# Autodesk Inventor assembly: Telaietto trasmissione - Taglio
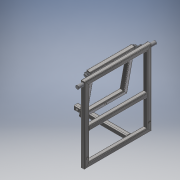
[picture p0: Inventor's stored thumbnail of the model, 180x180]
Saved by Autodesk Inventor 2018 (Build 220112000, 112)
## iProperties
Created: 2020-06-04
Part Number: Telaietto trasmissione - Taglio
Material: Generico
Document SubType Name: Weldment
Designer: Francesco
Weld Material: Welded Aluminum-6061
Mass: 1931.15 g
Surface Area: 2480.54 cm^2
Volume: 246.006 cm^3
Density: 7.85 g/cm^3
Author: Francesco
## Documents named in this file (10)
- C:\Users\Francesco\no-brim\Meccanica\Progetto Inventor no-brim\Assiemi\Telaietto trasmissione - Taglio.iam
- C:\Users\Francesco\no-brim\Meccanica\Progetto Inventor no-brim\Parti\Tubolare telaietto corto.ipt
- C:\Users\Francesco\no-brim\Meccanica\Progetto Inventor no-brim\Parti\Tubolare telaietto lungo 45.ipt
- C:\Users\Francesco\no-brim\Meccanica\Progetto Inventor no-brim\Parti\Tubolare telaietto corto 45.ipt
- C:\Users\Francesco\no-brim\Meccanica\Progetto Inventor no-brim\Parti\Tubolare telaietto corto 45 motore.ipt
- C:\Users\Francesco\no-brim\Meccanica\Progetto Inventor no-brim\Parti\Tubolare telaietto corto 45 motore per perni.ipt
- C:\Users\Francesco\no-brim\Meccanica\Progetto Inventor no-brim\Parti\Perno tendi motore.ipt
- C:\Users\Francesco\no-brim\Meccanica\Progetto Inventor no-brim\Parti\Supporto perno tendi motore.ipt
- C:\Users\Francesco\no-brim\Meccanica\Progetto Inventor no-brim\Parti\Perno movimento lama.ipt
- C:\Users\Francesco\no-brim\Meccanica\Progetto Inventor no-brim\Parti\Tubolare telaietto verticale.ipt
## Components (17 placed, 6 different names)
1. Tubolare telaietto corto:2 — Coincidente:8, Allineato:5, Coincidente:9
2. Tubolare telaietto lungo 45:1 — Coincidente:1, Allineato:1, Coincidente:2, Coincidente:5, Allineato:3, Coincidente:6, Coincidente:8, Allineato:5, Angolo:1, Coincidente:50, Coincidente:51, Allineato:20
3. Tubolare telaietto lungo 45:2 — Coincidente:3, Allineato:2, Coincidente:4, Allineato:18, Coincidente:48, Coincidente:49
4. Tubolare telaietto corto:3 — Coincidente:1, Allineato:1, Coincidente:2, Coincidente:3, Allineato:2, Coincidente:4, Coincidente:9, Coincidente:27, Coincidente:31, Allineato:14
5. Tubolare telaietto corto:4 — Coincidente:5, Allineato:3, Coincidente:6, Coincidente:52, Allineato:19
6. Perno tendi motore:1 — Coincidente:34, Coincidente:41
7. Perno tendi motore:2 — Coincidente:33, Coincidente:42, Coincidente:43
8. Supporto perno tendi motore:1 — Coincidente:31, Coincidente:33, Allineato:14, Coincidente:44
9. Supporto perno tendi motore:2 — Coincidente:27, Coincidente:34, Coincidente:47, Allineato:18
10. Tubolare telaietto corto:11 — Coincidente:35, Coincidente:36, Allineato:15, Coincidente:39, Allineato:17, Coincidente:40
11. Tubolare telaietto corto:12 — Coincidente:37, Allineato:16, Coincidente:38
12. Tubolare telaietto corto:13 — Coincidente:39, Allineato:17, Coincidente:40, Coincidente:45, Coincidente:46, Coincidente:47
13. Tubolare telaietto corto:14 — Coincidente:35, Coincidente:36, Allineato:15, Coincidente:37, Allineato:16, Coincidente:38, Coincidente:41, Coincidente:42, Coincidente:43, Coincidente:44, Angolo:1
14. Perno tendi motore:3 — Coincidente:45, Coincidente:46
15. Perno movimento lama:1 — Coincidente:48, Coincidente:49
16. Perno movimento lama:2 — Coincidente:50, Coincidente:51
17. Tubolare telaietto verticale:1 — Coincidente:52, Allineato:19, Allineato:20
## Relationships (42: Mate 30, Flush 11, Angle 1)
- Coincidente:1 [Mate]: Tubolare telaietto lungo 45:1 ↔ Tubolare telaietto corto:3
- Allineato:1 [Flush]: Tubolare telaietto lungo 45:1 ↔ Tubolare telaietto corto:3
- Coincidente:2 [Mate]: Tubolare telaietto lungo 45:1 ↔ Tubolare telaietto corto:3
- Coincidente:3 [Mate]: Tubolare telaietto lungo 45:2 ↔ Tubolare telaietto corto:3
- Allineato:2 [Flush]: Tubolare telaietto lungo 45:2 ↔ Tubolare telaietto corto:3
- Coincidente:4 [Mate]: Tubolare telaietto lungo 45:2 ↔ Tubolare telaietto corto:3
- Coincidente:5 [Mate]: Tubolare telaietto lungo 45:1 ↔ Tubolare telaietto corto:4
- Allineato:3 [Flush]: Tubolare telaietto lungo 45:1 ↔ Tubolare telaietto corto:4
- Coincidente:6 [Mate]: Tubolare telaietto lungo 45:1 ↔ Tubolare telaietto corto:4
- Coincidente:8 [Mate]: Tubolare telaietto corto:2 ↔ Tubolare telaietto lungo 45:1
- Allineato:5 [Flush]: Tubolare telaietto corto:2 ↔ Tubolare telaietto lungo 45:1
- Coincidente:9 [Mate] (-200 mm): Tubolare telaietto corto:2 ↔ Tubolare telaietto corto:3
- Coincidente:27 [Mate]: Tubolare telaietto corto:3 ↔ Supporto perno tendi motore:2
- Coincidente:31 [Mate]: Tubolare telaietto corto:3 ↔ Supporto perno tendi motore:1
- Coincidente:33 [Mate]: Perno tendi motore:2 ↔ Supporto perno tendi motore:1
- Coincidente:34 [Mate]: Perno tendi motore:1 ↔ Supporto perno tendi motore:2
- Allineato:14 [Flush]: Tubolare telaietto corto:3 ↔ Supporto perno tendi motore:1
- Coincidente:35 [Mate]: Tubolare telaietto corto:11 ↔ Tubolare telaietto corto:14
- Coincidente:36 [Mate]: Tubolare telaietto corto:11 ↔ Tubolare telaietto corto:14
- Allineato:15 [Flush]: Tubolare telaietto corto:11 ↔ Tubolare telaietto corto:14
- Coincidente:37 [Mate]: Tubolare telaietto corto:12 ↔ Tubolare telaietto corto:14
- Allineato:16 [Flush]: Tubolare telaietto corto:12 ↔ Tubolare telaietto corto:14
- Coincidente:38 [Mate]: Tubolare telaietto corto:12 ↔ Tubolare telaietto corto:14
- Coincidente:39 [Mate]: Tubolare telaietto corto:11 ↔ Tubolare telaietto corto:13
- Allineato:17 [Flush]: Tubolare telaietto corto:11 ↔ Tubolare telaietto corto:13
- Coincidente:40 [Mate]: Tubolare telaietto corto:11 ↔ Tubolare telaietto corto:13
- Coincidente:41 [Mate]: Perno tendi motore:1 ↔ Tubolare telaietto corto:14
- Coincidente:42 [Mate]: Perno tendi motore:2 ↔ Tubolare telaietto corto:14
- Coincidente:43 [Mate]: Perno tendi motore:2 ↔ Tubolare telaietto corto:14
- Coincidente:44 [Mate] (5 mm): Supporto perno tendi motore:1 ↔ Tubolare telaietto corto:14
- Coincidente:45 [Mate]: Tubolare telaietto corto:13 ↔ Perno tendi motore:3
- Coincidente:46 [Mate]: Tubolare telaietto corto:13 ↔ Perno tendi motore:3
- Coincidente:47 [Mate] (5 mm): Supporto perno tendi motore:2 ↔ Tubolare telaietto corto:13
- Allineato:18 [Flush] (25 mm): Tubolare telaietto lungo 45:2 ↔ Supporto perno tendi motore:2
- Angolo:1 [Angle] (190 deg): Tubolare telaietto lungo 45:1 ↔ Tubolare telaietto corto:14
- Coincidente:48 [Mate]: Tubolare telaietto lungo 45:2 ↔ Perno movimento lama:1
- Coincidente:49 [Mate]: Tubolare telaietto lungo 45:2 ↔ Perno movimento lama:1
- Coincidente:50 [Mate]: Tubolare telaietto lungo 45:1 ↔ Perno movimento lama:2
- Coincidente:51 [Mate]: Tubolare telaietto lungo 45:1 ↔ Perno movimento lama:2
- Coincidente:52 [Mate]: Tubolare telaietto corto:4 ↔ Tubolare telaietto verticale:1
- Allineato:19 [Flush]: Tubolare telaietto corto:4 ↔ Tubolare telaietto verticale:1
- Allineato:20 [Flush] (74 mm): Tubolare telaietto lungo 45:1 ↔ Tubolare telaietto verticale:1
